# Autodesk Inventor assembly: pitahaya
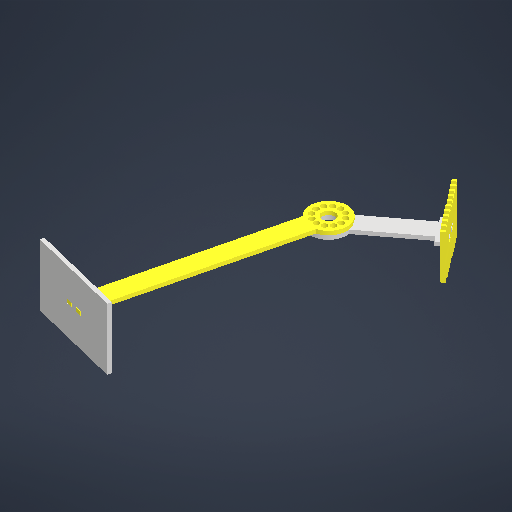
[picture p0: Inventor's stored thumbnail of the model, 512x512]
Saved by Autodesk Inventor 2026.3 (Build 303398000, 398)
## iProperties
Created: 2026-09-15
Part Number: pitahaya
Document SubType Name: Assembly
Designer: micha
Author: micha
## Documents named in this file (5)
- C:\Projects\startup\Espressif\esp32-cam-pitahaya\autodesk\pitahaya.iam
- C:\Projects\startup\Espressif\esp32-cam-pitahaya\autodesk\pitahaya1.ipt
- C:\Projects\startup\Espressif\esp32-cam-pitahaya\autodesk\pitahaya2.ipt
- C:\Projects\startup\Espressif\esp32-cam-pitahaya\autodesk\pitahaya3.ipt
- C:\Projects\startup\Espressif\esp32-cam-pitahaya\autodesk\pitahaya4.ipt
## Components (4 placed, 4 different names)
1. pitahaya1:1 — Mate:2, Mate:3, Mate:4, Mate:5, Flush:1
2. pitahaya2:1 — Mate:2, Mate:3, Mate:6, Mate:7, Mate:8
3. pitahaya3:1 — Mate:4, Mate:5, Flush:1
4. pitahaya4:1 — Mate:6, Mate:7, Mate:8
## Relationships (8: Mate 7, Flush 1)
- Mate:2: pitahaya1:1 ↔ pitahaya2:1
- Mate:3: pitahaya1:1 ↔ pitahaya2:1
- Mate:4: pitahaya1:1 ↔ pitahaya3:1
- Mate:5: pitahaya1:1 ↔ pitahaya3:1
- Flush:1: pitahaya1:1 ↔ pitahaya3:1
- Mate:6: pitahaya2:1 ↔ pitahaya4:1
- Mate:7: pitahaya2:1 ↔ pitahaya4:1
- Mate:8: pitahaya2:1 ↔ pitahaya4:1
